# Autodesk Inventor assembly: Idler
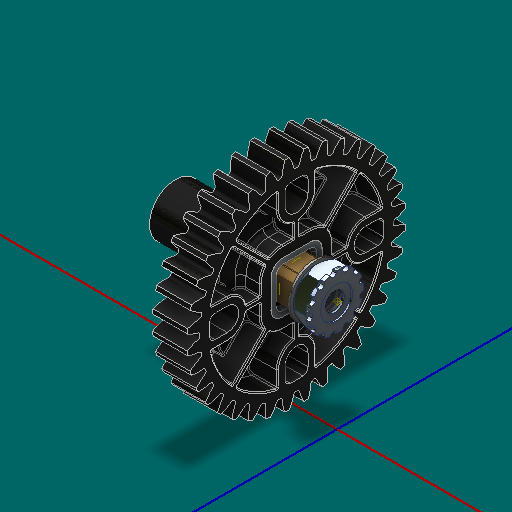
[picture p0: Inventor's stored thumbnail of the model, 512x512]
Saved by Autodesk Inventor 2025 (Build 290162000, 162)
## iProperties
Created: 2024-10-18
Part Number: Idler
Document SubType Name: Assembly
Designer: averey
Author: averey
## Documents named in this file (8)
- C:\Users\avere\VEX\High Stakes\CAD\V2\Chassis\Drivebay Left\Idler.iam
- C:\Users\avere\vex_robotics_high_stakes\hardware\cad\robpros_cad_lib\Motion\Spacers\Washer Steel\SWasher .375 OD x .015625.ipt
- C:\Users\avere\vex_robotics_high_stakes\hardware\cad\robpros_cad_lib\Motion\Spacers\Washer Steel.ipt
- C:\Users\avere\vex_robotics_high_stakes\hardware\cad\robpros_cad_lib\Modified Parts\modified_parts\Half Cut HS 36T Gear, No Insert.ipt
- C:\Users\avere\vex_robotics_high_stakes\hardware\cad\robpros_cad_lib\Motion\HS Shaft Adapter Circle.ipt
- C:\Users\avere\vex_robotics_high_stakes\hardware\cad\robpros_cad_lib\Structure\Hardware\Nut Keps.ipt
- C:\Users\avere\vex_robotics_high_stakes\hardware\cad\VEX-CAD-Inventor\Motion\Spacers\Spacer Nylon .375 OD\NSpacer .375 OD x .500.ipt
- C:\Users\avere\vex_robotics_high_stakes\hardware\cad\VEX-CAD-Inventor\Motion\Spacers\Spacer Nylon .375 OD.ipt
## Components (5 placed, 5 different names)
1. Half Cut HS 36T Gear, No Insert:1
2. HS Shaft Adapter Circle:1
3. Nut Keps:1 — Mate:1
4. SWasher .375 OD x .015625:1
5. NSpacer .375 OD x .500:1
## Relationships (6: Insert 4, Angle 1, Mate 1)
- [Insert] (-3.175 mm): Half Cut HS 36T Gear, No Insert:1 ↔ HS Shaft Adapter Circle:1
- [Angle] (0 deg): Half Cut HS 36T Gear, No Insert:1 ↔ HS Shaft Adapter Circle:1
- [Insert] (3.175 mm): Half Cut HS 36T Gear, No Insert:1 ↔ SWasher .375 OD x .015625:1
- [Insert]: HS Shaft Adapter Circle:1 ↔ NSpacer .375 OD x .500:1
- [Insert]: Nut Keps:1 ↔ SWasher .375 OD x .015625:1
- Mate:1: Nut Keps:1
## Named parameters: d6_d7 = 3.175 mm
